# Autodesk Inventor assembly: BB-42016_MIR1
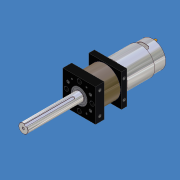
[picture p0: Inventor's stored thumbnail of the model, 180x180]
Saved by Autodesk Inventor 2015 (Build 190159000, 159)
## iProperties
Created: 2007-01-14
Part Number: BB-42016_MIR1
Catalog Web Link: www.banebots.com
Description: BaneBots 42mm Gearbox 16:1
Vendor: BaneBots
Document SubType Name: Assembly
Designer: whitaus15
Company: FirstCadLibrary
Title: BaneBots 42mm Gearbox 16:1
Author: Ed Sparks
## Documents named in this file (7)
- \\lhssvr02\Homedirs\Robotics Club\CAD Model 2015\Parts Folder\Gear Boxes\Bane Bots\16-1\BB-42016_MIR1.iam
- \\lhssvr02\Homedirs\Robotics Club\CAD Model 2015\Parts Folder\Gear Boxes\Bane Bots\16-1\BB5-FrontPlate_MIR1.ipt
- \\lhssvr02\Homedirs\Robotics Club\CAD Model 2015\Parts Folder\Gear Boxes\Bane Bots\16-1\BB5-Bearing_MIR1.ipt
- \\lhssvr02\Homedirs\Robotics Club\CAD Model 2015\Parts Folder\Gear Boxes\Bane Bots\16-1\BB5-Axle_MIR1.ipt
- \\lhssvr02\Homedirs\Robotics Club\CAD Model 2015\Parts Folder\Gear Boxes\Bane Bots\16-1\BB5-RingGear_MIR1.ipt
- \\lhssvr02\Homedirs\Robotics Club\CAD Model 2015\Parts Folder\Gear Boxes\Bane Bots\16-1\BB5-BackPlate_MIR1.ipt
- \\lhssvr02\Homedirs\Robotics Club\CAD Model 2015\Parts Folder\Gear Boxes\Bane Bots\16-1\FisherPriceMotor_MIR1.ipt
## Components (7 placed, 6 different names)
1. BB5-FrontPlate_MIR1:1 — Flush:1, Mate:3, Mate:8, Mate:7, Mate:6
2. BB5-Bearing_MIR1:1 — Flush:1, Mate:3, Mate:5, Mate:4, Mate:2, Mate:1
3. BB5-Bearing_MIR1:2 — Mate:2, Mate:1
4. BB5-Axle_MIR1:1 — Mate:5, Mate:4
5. BB5-RingGear_MIR1:1 — Mate:8, Mate:7, Mate:6, Mate:11, Mate:10, Mate:9
6. BB5-BackPlate_MIR1:1 — Mate:11, Mate:10, Mate:9, Mate:14, Mate:13, Mate:12
7. FisherPriceMotor_MIR1:1 — Mate:14, Mate:13, Mate:12
## Relationships (15: Mate 14, Flush 1)
- Flush:1: BB5-FrontPlate_MIR1:1 ↔ BB5-Bearing_MIR1:1
- Mate:3: BB5-FrontPlate_MIR1:1 ↔ BB5-Bearing_MIR1:1
- Mate:5: BB5-Bearing_MIR1:1 ↔ BB5-Axle_MIR1:1
- Mate:4: BB5-Bearing_MIR1:1 ↔ BB5-Axle_MIR1:1
- Mate:8: BB5-FrontPlate_MIR1:1 ↔ BB5-RingGear_MIR1:1
- Mate:7: BB5-FrontPlate_MIR1:1 ↔ BB5-RingGear_MIR1:1
- Mate:6: BB5-FrontPlate_MIR1:1 ↔ BB5-RingGear_MIR1:1
- Mate:11: BB5-RingGear_MIR1:1 ↔ BB5-BackPlate_MIR1:1
- Mate:10: BB5-RingGear_MIR1:1 ↔ BB5-BackPlate_MIR1:1
- Mate:9: BB5-RingGear_MIR1:1 ↔ BB5-BackPlate_MIR1:1
- Mate:14: BB5-BackPlate_MIR1:1 ↔ FisherPriceMotor_MIR1:1
- Mate:13: BB5-BackPlate_MIR1:1 ↔ FisherPriceMotor_MIR1:1
- Mate:12: BB5-BackPlate_MIR1:1 ↔ FisherPriceMotor_MIR1:1
- Mate:2: BB5-Bearing_MIR1:1 ↔ BB5-Bearing_MIR1:2
- Mate:1: BB5-Bearing_MIR1:1 ↔ BB5-Bearing_MIR1:2
